# Autodesk Inventor assembly: X-End-Idler v0.1
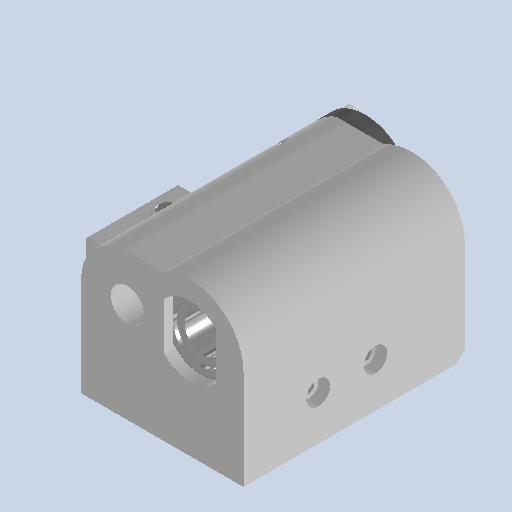
[picture p0: Inventor's stored thumbnail of the model, 512x512]
Saved by Autodesk Inventor 2023 (Build 270158000, 158)
## iProperties
Created: 2023-07-26
Part Number: X-End-Idler v0.1
Document SubType Name: Assembly
Designer: Parker
Mass: 195.319 g
Surface Area: 399.977 cm^2
Volume: 92.2149 cm^3
Density: 2.11808 g/cm^3
Author: Parker
## Documents named in this file (13)
- D:\000 - PEPCORP CLOUD\00- Legacy\Designs\MK3PRO P1\X-Axis\X-End-Idler v0.1.iam
- D:\000 - PEPCORP CLOUD\00- Legacy\Designs\MK3PRO P1\X-Axis\X-End-Idler v0.3.ipt
- X-End-Idler v0.4.ipt
- D:\000 - PEPCORP CLOUD\00- Legacy\Designs\MK3PRO P1\COMPONENTS\Idler Roller, flat.ipt
- D:\000 - PEPCORP CLOUD\00- Legacy\Designs\MK3PRO P1\X-Axis\X-End-Floating-Idler v0.1.ipt
- X-End-Floating-Idler v0.4.ipt
- D:\000 - PEPCORP CLOUD\00- Legacy\Designs\MK3PRO P1\COMPONENTS\SHCS_M3_25.ipt
- D:\000 - PEPCORP CLOUD\00- Legacy\Designs\MK3PRO P1\COMPONENTS\M5 Nylock.ipt
- D:\000 - PEPCORP CLOUD\00- Legacy\Designs\MK3PRO P1\X-Axis\Z_NUT_1.ipt
- D:\000 - PEPCORP CLOUD\00- Legacy\Designs\MK3PRO P1\COMPONENTS\NUT_SQUARE_M3.ipt
- D:\000 - PEPCORP CLOUD\00- Legacy\Designs\MK3PRO P1\COMPONENTS\SHCS_M3_18.ipt
- D:\000 - PEPCORP CLOUD\00- Legacy\Designs\MK3PRO P1\COMPONENTS\LM10UU.ipt
- C:\Users\Parker\Documents\Inventor\Content Center Files\R2023\en-US\JIS B 1174\JIS B 1174 - M5 x 25.ipt
## Components (16 placed, 10 different names)
1. X-End-Idler v0.4:1 — Mate:1, Mate:15, Mate:16, Mate:21, Mate:22, Angle:3, Angle:4, Mate:23, Mate:24, Mate:25, Mate:26, Mate:31, Mate:32, Mate:33, Mate:35, Mate:36, Mate:37, Mate:38, Mate:39
2. Idler Roller, flat:1 — Mate:8, Mate:9, Mate:42
3. X-End-Floating-Idler v0.4:1 — Mate:1, Mate:8, Mate:9, Mate:12, Mate:17, Mate:18, Mate:19, Mate:20, Angle:1, Angle:2, Mate:39, Mate:41, Mate:43
4. SHCS_M3_25:1 — Mate:36, Mate:38
5. SHCS_M3_25:2 — Mate:35, Mate:37, Mate:41
6. M5 Nylock:1 — Mate:12, Mate:44
7. Z_NUT_1:1 — Mate:23, Mate:24, Mate:25, Mate:26, Mate:27, Mate:28, Mate:29, Mate:30
8. NUT_SQUARE_M3:1 — Mate:17, Mate:20, Angle:1
9. NUT_SQUARE_M3:2 — Mate:16, Mate:21, Angle:4
10. NUT_SQUARE_M3:3 — Mate:18, Mate:19, Angle:2
11. NUT_SQUARE_M3:4 — Mate:15, Mate:22, Angle:3
12. SHCS_M3_18:1 — Mate:28, Mate:29
13. SHCS_M3_18:2 — Mate:27, Mate:30
14. LM10UU:1 — Mate:31, Mate:32, Mate:34
15. LM10UU:2 — Mate:33, Mate:34
16. JIS B 1174 - Metric M5 x 25:1 — Mate:42, Mate:43, Mate:44
## Relationships (37: Mate 33, Angle 4)
- Mate:1 (1 mm): X-End-Idler v0.4:1 ↔ X-End-Floating-Idler v0.4:1
- Mate:8: Idler Roller, flat:1 ↔ X-End-Floating-Idler v0.4:1
- Mate:9: Idler Roller, flat:1 ↔ X-End-Floating-Idler v0.4:1
- Mate:12: X-End-Floating-Idler v0.4:1 ↔ M5 Nylock:1
- Mate:15: X-End-Idler v0.4:1 ↔ NUT_SQUARE_M3:4
- Mate:16: X-End-Idler v0.4:1 ↔ NUT_SQUARE_M3:2
- Mate:17: X-End-Floating-Idler v0.4:1 ↔ NUT_SQUARE_M3:1
- Mate:18: X-End-Floating-Idler v0.4:1 ↔ NUT_SQUARE_M3:3
- Mate:19: X-End-Floating-Idler v0.4:1 ↔ NUT_SQUARE_M3:3
- Mate:20: X-End-Floating-Idler v0.4:1 ↔ NUT_SQUARE_M3:1
- Angle:1 (0 deg): X-End-Floating-Idler v0.4:1 ↔ NUT_SQUARE_M3:1
- Angle:2 (0 deg): X-End-Floating-Idler v0.4:1 ↔ NUT_SQUARE_M3:3
- Mate:21: X-End-Idler v0.4:1 ↔ NUT_SQUARE_M3:2
- Mate:22: X-End-Idler v0.4:1 ↔ NUT_SQUARE_M3:4
- Angle:3 (0 deg): X-End-Idler v0.4:1 ↔ NUT_SQUARE_M3:4
- Angle:4 (0 deg): X-End-Idler v0.4:1 ↔ NUT_SQUARE_M3:2
- Mate:23: X-End-Idler v0.4:1 ↔ Z_NUT_1:1
- Mate:24: X-End-Idler v0.4:1 ↔ Z_NUT_1:1
- Mate:25: X-End-Idler v0.4:1 ↔ Z_NUT_1:1
- Mate:26: X-End-Idler v0.4:1 ↔ Z_NUT_1:1
- Mate:27: Z_NUT_1:1 ↔ SHCS_M3_18:2
- Mate:28: Z_NUT_1:1 ↔ SHCS_M3_18:1
- Mate:29: Z_NUT_1:1 ↔ SHCS_M3_18:1
- Mate:30: Z_NUT_1:1 ↔ SHCS_M3_18:2
- Mate:31: X-End-Idler v0.4:1 ↔ LM10UU:1
- Mate:32: X-End-Idler v0.4:1 ↔ LM10UU:1
- Mate:33: X-End-Idler v0.4:1 ↔ LM10UU:2
- Mate:34: LM10UU:1 ↔ LM10UU:2
- Mate:35: X-End-Idler v0.4:1 ↔ SHCS_M3_25:2
- Mate:36: X-End-Idler v0.4:1 ↔ SHCS_M3_25:1
- Mate:37: X-End-Idler v0.4:1 ↔ SHCS_M3_25:2
- Mate:38: X-End-Idler v0.4:1 ↔ SHCS_M3_25:1
- Mate:39: X-End-Idler v0.4:1 ↔ X-End-Floating-Idler v0.4:1
- Mate:41: X-End-Floating-Idler v0.4:1 ↔ SHCS_M3_25:2
- Mate:42: Idler Roller, flat:1 ↔ JIS B 1174 - Metric M5 x 25:1
- Mate:43: X-End-Floating-Idler v0.4:1 ↔ JIS B 1174 - Metric M5 x 25:1
- Mate:44: M5 Nylock:1 ↔ JIS B 1174 - Metric M5 x 25:1
